# Autodesk Inventor assembly: Tape Winch
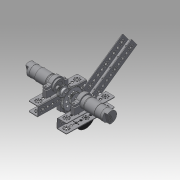
[picture p0: Inventor's stored thumbnail of the model, 180x180]
Saved by Autodesk Inventor 2016 (Build 200138000, 138)
## iProperties
Created: 2016-02-10
Part Number: Tape Winch
Document SubType Name: Assembly
Designer: Delta
Author: Delta
## Documents named in this file (14)
- C:\Robotics\CAD\2015-16\custom cad parts\Tape Winch.iam
- C:\Robotics\CAD\2015-16\COTSParts\Tetrix\Tetrix channel 160mm.ipt
- C:\Robotics\CAD\2015-16\COTSParts\Tetrix\Tetrix Gear 80T.ipt
- C:\Robotics\CAD\2015-16\COTSParts\Tetrix\Tetrix Hub - axle.ipt
- C:\Robotics\CAD\2015-16\COTSParts\Tetrix\Tetrix motor mount.ipt
- C:\Robotics\CAD\2015-16\COTSParts\Motors\Andymark 2964  NeveRest 40 Motor.ipt
- C:\Robotics\CAD\2015-16\COTSParts\Tetrix\Tetrix Gear 40T.ipt
- C:\Robotics\CAD\2015-16\custom cad parts\Foam Wheel.ipt
- C:\Robotics\CAD\2015-16\custom cad parts\Tape speel cylinder.ipt
- C:\Robotics\CAD\2015-16\COTSParts\Tetrix\Tetrix shaft 100mm_MIR2.ipt
- C:\Robotics\CAD\2015-16\COTSParts\Tetrix\Bronze bushing_MIR2.ipt
- C:\Robotics\CAD\2015-16\COTSParts\Tetrix\Nylon spacer - large_MIR2.ipt
- C:\Robotics\CAD\2015-16\COTSParts\Tetrix\Nylon spacer - small.ipt
- C:\Robotics\CAD\2015-16\COTSParts\Tetrix\Tetrix motor_MIR2.ipt
## Components (24 placed, 13 different names)
1. Tetrix channel 160mm:1 — Mate:2, Mate:3
2. Tetrix channel 160mm:2 — Mate:1, Flush:1, Flush:2, Mate:2, Mate:3, Mate:4, Mate:6, Mate:13, Mate:14, Mate:15, Mate:21, Mate:22, Mate:23, Mate:41, Mate:42
3. Tetrix channel 160mm:3 — Mate:1, Flush:1, Flush:2, Mate:5, Mate:7, Mate:10, Mate:11, Mate:12, Mate:39, Mate:46
4. Tetrix Gear 80T:1 — Mate:5, Mate:7, Flush:6, Mate:27, Mate:32
5. Tetrix Gear 80T:2 — Mate:4, Mate:6, Mate:8, Mate:9, Flush:5, Mate:36
6. Tetrix Hub - axle:1 — Mate:8, Mate:9
7. Tetrix motor mount:1 — Mate:10, Mate:11, Mate:12, Mate:16, Flush:3
8. Tetrix motor mount:2 — Mate:13, Mate:14, Mate:15, Mate:18, Flush:4
9. Andymark 2964  NeveRest 40 Motor:1 — Mate:16, Flush:3, Mate:17, Mate:20, Mate:31
10. Andymark 2964  NeveRest 40 Motor:2 — Mate:17, Mate:18, Flush:4, Mate:19, Mate:29
11. Tetrix Gear 40T:1 — Mate:20, Flush:6, Mate:28, Mate:34
12. Tetrix Gear 40T:2 — Mate:19, Flush:5, Mate:28, Mate:30, Mate:35
13. Tetrix motor mount:3 — Mate:21, Mate:22, Mate:23, Mate:47
14. Foam Wheel:1 — Mate:27, Flush:8, Mate:48, Mate:49
15. Tetrix Hub - axle:2 — Mate:29, Mate:30, Mate:33, Mate:35
16. Tetrix Hub - axle:3 — Mate:31, Mate:32, Mate:33, Mate:34
17. Tape speel cylinder:1 — Mate:36, Flush:8, Mate:37
18. Tetrix shaft 100mm_MIR2:1 — Mate:37, Mate:38, Mate:40
19. Bronze bushing_MIR2:1 — Mate:38, Mate:39
20. Bronze bushing_MIR2:2 — Mate:40, Mate:41
21. Nylon spacer - large_MIR2:1 — Mate:42, Mate:43, Mate:46
22. Nylon spacer - large_MIR2:2 — Mate:43, Mate:44, Mate:45
23. Nylon spacer - small:1 — Mate:44, Mate:45
24. Tetrix motor_MIR2:1 — Mate:47, Mate:48, Mate:49
## Relationships (53: Mate 46, Flush 7)
- Mate:1 (63.5 mm): Tetrix channel 160mm:2 ↔ Tetrix channel 160mm:3
- Flush:1: Tetrix channel 160mm:2 ↔ Tetrix channel 160mm:3
- Flush:2: Tetrix channel 160mm:2 ↔ Tetrix channel 160mm:3
- Mate:2 (19.558 mm): Tetrix channel 160mm:1 ↔ Tetrix channel 160mm:2
- Mate:3: Tetrix channel 160mm:1 ↔ Tetrix channel 160mm:2
- Mate:4 (12 mm): Tetrix channel 160mm:2 ↔ Tetrix Gear 80T:2
- Mate:5 (4 mm): Tetrix channel 160mm:3 ↔ Tetrix Gear 80T:1
- Mate:6: Tetrix channel 160mm:2 ↔ Tetrix Gear 80T:2
- Mate:7: Tetrix channel 160mm:3 ↔ Tetrix Gear 80T:1
- Mate:8: Tetrix Gear 80T:2 ↔ Tetrix Hub - axle:1
- Mate:9: Tetrix Gear 80T:2 ↔ Tetrix Hub - axle:1
- Mate:10: Tetrix channel 160mm:3 ↔ Tetrix motor mount:1
- Mate:11: Tetrix channel 160mm:3 ↔ Tetrix motor mount:1
- Mate:12: Tetrix channel 160mm:3 ↔ Tetrix motor mount:1
- Mate:13: Tetrix channel 160mm:2 ↔ Tetrix motor mount:2
- Mate:14: Tetrix channel 160mm:2 ↔ Tetrix motor mount:2
- Mate:15: Tetrix channel 160mm:2 ↔ Tetrix motor mount:2
- Mate:16: Tetrix motor mount:1 ↔ Andymark 2964  NeveRest 40 Motor:1
- Flush:3 (-2 mm): Tetrix motor mount:1 ↔ Andymark 2964  NeveRest 40 Motor:1
- Mate:17: Andymark 2964  NeveRest 40 Motor:1 ↔ Andymark 2964  NeveRest 40 Motor:2
- Mate:18: Tetrix motor mount:2 ↔ Andymark 2964  NeveRest 40 Motor:2
- Flush:4 (6 mm): Tetrix motor mount:2 ↔ Andymark 2964  NeveRest 40 Motor:2
- Mate:19: Andymark 2964  NeveRest 40 Motor:2 ↔ Tetrix Gear 40T:2
- Mate:20: Andymark 2964  NeveRest 40 Motor:1 ↔ Tetrix Gear 40T:1
- Flush:5: Tetrix Gear 80T:2 ↔ Tetrix Gear 40T:2
- Flush:6: Tetrix Gear 80T:1 ↔ Tetrix Gear 40T:1
- Mate:21: Tetrix channel 160mm:2 ↔ Tetrix motor mount:3
- Mate:22: Tetrix channel 160mm:2 ↔ Tetrix motor mount:3
- Mate:23: Tetrix channel 160mm:2 ↔ Tetrix motor mount:3
- Mate:27 (3.2639 mm): Tetrix Gear 80T:1 ↔ Foam Wheel:1
- Mate:28: Tetrix Gear 40T:1 ↔ Tetrix Gear 40T:2
- Mate:29: Andymark 2964  NeveRest 40 Motor:2 ↔ Tetrix Hub - axle:2
- Mate:30: Tetrix Gear 40T:2 ↔ Tetrix Hub - axle:2
- Mate:31: Andymark 2964  NeveRest 40 Motor:1 ↔ Tetrix Hub - axle:3
- Mate:32: Tetrix Gear 80T:1 ↔ Tetrix Hub - axle:3
- Mate:33: Tetrix Hub - axle:2 ↔ Tetrix Hub - axle:3
- Mate:34: Tetrix Gear 40T:1 ↔ Tetrix Hub - axle:3
- Mate:35: Tetrix Gear 40T:2 ↔ Tetrix Hub - axle:2
- Mate:36: Tetrix Gear 80T:2 ↔ Tape speel cylinder:1
- Flush:8: Foam Wheel:1 ↔ Tape speel cylinder:1
- Mate:37: Tape speel cylinder:1 ↔ Tetrix shaft 100mm_MIR2:1
- Mate:38: Tetrix shaft 100mm_MIR2:1 ↔ Bronze bushing_MIR2:1
- Mate:39: Tetrix channel 160mm:3 ↔ Bronze bushing_MIR2:1
- Mate:40: Tetrix shaft 100mm_MIR2:1 ↔ Bronze bushing_MIR2:2
- Mate:41: Tetrix channel 160mm:2 ↔ Bronze bushing_MIR2:2
- Mate:42: Tetrix channel 160mm:2 ↔ Nylon spacer - large_MIR2:1
- Mate:43: Nylon spacer - large_MIR2:1 ↔ Nylon spacer - large_MIR2:2
- Mate:44: Nylon spacer - large_MIR2:2 ↔ Nylon spacer - small:1
- Mate:45: Nylon spacer - large_MIR2:2 ↔ Nylon spacer - small:1
- Mate:46: Tetrix channel 160mm:3 ↔ Nylon spacer - large_MIR2:1
- Mate:47: Tetrix motor mount:3 ↔ Tetrix motor_MIR2:1
- Mate:48: Foam Wheel:1 ↔ Tetrix motor_MIR2:1
- Mate:49 (15.24 mm): Foam Wheel:1 ↔ Tetrix motor_MIR2:1
